# Autodesk Inventor assembly: Layout Test Assembly
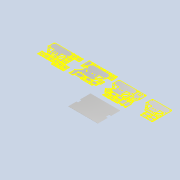
[picture p0: Inventor's stored thumbnail of the model, 180x180]
Saved by Autodesk Inventor 2022 (Build 260153000, 153)
## iProperties
Created: 2021-10-30
Part Number: Layout Test Assembly
Document SubType Name: Assembly
Designer: Coy
Author: Coy
## Documents named in this file (12)
- H:\3D Files\Project 3D Models\Breakfast Maker 2000\Machined Parts\Layout Test Assembly.iam
- H:\3D Files\Project 3D Models\Breakfast Maker 2000\Machined Parts\Stock Aluminum Sheet.ipt
- H:\3D Files\Project 3D Models\Breakfast Maker 2000\Machined Parts\X Axis Belt Motor Inside Frame Machined.ipt
- H:\3D Files\Project 3D Models\Breakfast Maker 2000\Machined Parts\X Axis Belt V Wheel and Motor Frame Machined.ipt
- H:\3D Files\Project 3D Models\Breakfast Maker 2000\Machined Parts\X Axis Belt V Wheel Frame Machined.ipt
- H:\3D Files\Project 3D Models\Breakfast Maker 2000\Machined Parts\X Axis Belt V Wheel LEFT Outside Frame Machined.ipt
- H:\3D Files\Project 3D Models\Breakfast Maker 2000\Machined Parts\X Axis Belt V Wheel RIGHT Outside Frame Machined.ipt
- H:\3D Files\Project 3D Models\Breakfast Maker 2000\Machined Parts\2x4 2020 Extrusion Gusset Connector.ipt
- H:\3D Files\Project 3D Models\Breakfast Maker 2000\Machined Parts\X Axis Statonary Composite Belt Holder.ipt
- H:\3D Files\Project 3D Models\Breakfast Maker 2000\Machined Parts\X Axis Statonary NON ADJUSTABLE Composite Belt Holder.ipt
- H:\3D Files\Project 3D Models\Breakfast Maker 2000\Machined Parts\X Axis Drag Chain 2020 Connecting Bracket.ipt
- H:\3D Files\Project 3D Models\Breakfast Maker 2000\Machined Parts\Generic 3x3 Corner Connecting Gusset.ipt
## Components (34 placed, 11 different names)
1. Stock Aluminum Sheet:1 — Mate:1, Mate:2, Mate:3, Mate:4, Mate:5, Mate:6, Mate:7, Mate:8, Mate:9, Mate:10, Mate:11, Mate:12, Mate:13, Mate:14, Mate:15, Mate:16, Mate:17, Mate:18, Mate:19, Mate:20, Mate:22, Mate:23, Mate:24, Mate:26, Mate:28, Mate:29, Mate:30, Mate:31, Mate:42, Mate:54, Mate:55, Mate:84, Mate:85
2. X Axis Belt Motor Inside Frame Machined:1 — Mate:54, Mate:56, Flush:4, Mate:67
3. X Axis Belt V Wheel and Motor Frame Machined:1 — Mate:4, Mate:68, Flush:10, Flush:15, Mate:78, Mate:83
4. X Axis Belt V Wheel Frame Machined:1 — Mate:3, Mate:80, Mate:86, Flush:20
5. X Axis Belt V Wheel LEFT Outside Frame Machined:1 — Mate:2, Mate:56, Flush:4, Mate:57, Mate:58, Mate:64, Mate:81
6. X Axis Belt V Wheel RIGHT Outside Frame Machined:1 — Mate:1, Mate:43, Mate:44, Mate:45, Mate:46, Mate:48, Mate:51, Flush:2, Mate:52, Flush:3, Tangent:1, Mate:82
7. 2x4 2020 Extrusion Gusset Connector:1 — Mate:22, Mate:58, Mate:59, Mate:60, Mate:61, Mate:64, Tangent:3, Mate:65
8. 2x4 2020 Extrusion Gusset Connector:2 — Mate:23, Mate:47, Mate:48, Mate:49, Mate:50
9. X Axis Statonary Composite Belt Holder:1 — Mate:55, Mate:66, Flush:5
10. X Axis Statonary Composite Belt Holder:2 — Mate:24, Mate:65, Mate:66, Flush:5, Mate:67
11. X Axis Statonary NON ADJUSTABLE Composite Belt Holder:1 — Mate:26, Mate:43, Flush:1
12. X Axis Statonary NON ADJUSTABLE Composite Belt Holder:2 — Mate:42, Mate:45, Mate:46, Mate:47, Tangent:2
13. X Axis Drag Chain 2020 Connecting Bracket:1 — Mate:28, Mate:44, Flush:1, Flush:3, Mate:53
14. X Axis Drag Chain 2020 Connecting Bracket:2 — Mate:30, Mate:52, Mate:53
15. X Axis Drag Chain 2020 Connecting Bracket:3 — Mate:29, Mate:79, Flush:18
16. X Axis Drag Chain 2020 Connecting Bracket:4 — Mate:31, Mate:49, Tangent:2
17. Generic 3x3 Corner Connecting Gusset:1 — Mate:17, Mate:57, Tangent:3, Tangent:4
18. Generic 3x3 Corner Connecting Gusset:2 — Mate:18, Flush:12, Mate:75, Flush:17, Mate:77
19. Generic 3x3 Corner Connecting Gusset:3 — Mate:19, Flush:7, Flush:8, Mate:68, Mate:71, Mate:72
20. Generic 3x3 Corner Connecting Gusset:4 — Mate:20, Flush:6, Mate:70
21. Generic 3x3 Corner Connecting Gusset:5 — Mate:13, Flush:17, Mate:77, Mate:79, Flush:18
22. Generic 3x3 Corner Connecting Gusset:6 — Mate:14, Flush:16, Mate:76
23. Generic 3x3 Corner Connecting Gusset:7 — Mate:15, Mate:61, Mate:63
24. Generic 3x3 Corner Connecting Gusset:8 — Mate:16, Mate:51, Flush:2
25. Generic 3x3 Corner Connecting Gusset:9 — Mate:9, Flush:8, Mate:72, Flush:10
26. Generic 3x3 Corner Connecting Gusset:10 — Mate:10, Flush:13, Flush:14, Mate:73, Mate:74, Mate:78
27. Generic 3x3 Corner Connecting Gusset:11 — Mate:11, Flush:6, Flush:7, Mate:70, Mate:71
28. Generic 3x3 Corner Connecting Gusset:12 — Mate:12, Mate:50, Tangent:1
29. Generic 3x3 Corner Connecting Gusset:13 — Mate:5, Mate:60, Mate:62, Mate:63
30. Generic 3x3 Corner Connecting Gusset:14 — Mate:6, Mate:59, Mate:62, Tangent:4
31. Generic 3x3 Corner Connecting Gusset:15 — Mate:7, Flush:14, Mate:73, Flush:15, Flush:16, Mate:76
32. Generic 3x3 Corner Connecting Gusset:16 — Mate:8, Flush:12, Flush:13, Mate:74, Mate:75
33. 2x4 2020 Extrusion Gusset Connector:3 — Mate:85, Mate:87, Flush:19
34. 2x4 2020 Extrusion Gusset Connector:4 — Mate:84, Mate:86, Mate:87, Flush:19, Flush:20
## Relationships (95: Mate 73, Flush 18, Tangent 4)
- Mate:1: Stock Aluminum Sheet:1 ↔ X Axis Belt V Wheel RIGHT Outside Frame Machined:1
- Mate:2: Stock Aluminum Sheet:1 ↔ X Axis Belt V Wheel LEFT Outside Frame Machined:1
- Mate:3: Stock Aluminum Sheet:1 ↔ X Axis Belt V Wheel Frame Machined:1
- Mate:4: Stock Aluminum Sheet:1 ↔ X Axis Belt V Wheel and Motor Frame Machined:1
- Mate:5: Stock Aluminum Sheet:1 ↔ Generic 3x3 Corner Connecting Gusset:13
- Mate:6: Stock Aluminum Sheet:1 ↔ Generic 3x3 Corner Connecting Gusset:14
- Mate:7: Stock Aluminum Sheet:1 ↔ Generic 3x3 Corner Connecting Gusset:15
- Mate:8: Stock Aluminum Sheet:1 ↔ Generic 3x3 Corner Connecting Gusset:16
- Mate:9: Stock Aluminum Sheet:1 ↔ Generic 3x3 Corner Connecting Gusset:9
- Mate:10: Stock Aluminum Sheet:1 ↔ Generic 3x3 Corner Connecting Gusset:10
- Mate:11: Stock Aluminum Sheet:1 ↔ Generic 3x3 Corner Connecting Gusset:11
- Mate:12: Stock Aluminum Sheet:1 ↔ Generic 3x3 Corner Connecting Gusset:12
- Mate:13: Stock Aluminum Sheet:1 ↔ Generic 3x3 Corner Connecting Gusset:5
- Mate:14: Stock Aluminum Sheet:1 ↔ Generic 3x3 Corner Connecting Gusset:6
- Mate:15: Stock Aluminum Sheet:1 ↔ Generic 3x3 Corner Connecting Gusset:7
- Mate:16: Stock Aluminum Sheet:1 ↔ Generic 3x3 Corner Connecting Gusset:8
- Mate:17: Stock Aluminum Sheet:1 ↔ Generic 3x3 Corner Connecting Gusset:1
- Mate:18: Stock Aluminum Sheet:1 ↔ Generic 3x3 Corner Connecting Gusset:2
- Mate:19: Stock Aluminum Sheet:1 ↔ Generic 3x3 Corner Connecting Gusset:3
- Mate:20: Stock Aluminum Sheet:1 ↔ Generic 3x3 Corner Connecting Gusset:4
- Mate:22: Stock Aluminum Sheet:1 ↔ 2x4 2020 Extrusion Gusset Connector:1
- Mate:23: Stock Aluminum Sheet:1 ↔ 2x4 2020 Extrusion Gusset Connector:2
- Mate:24: Stock Aluminum Sheet:1 ↔ X Axis Statonary Composite Belt Holder:2
- Mate:26: Stock Aluminum Sheet:1 ↔ X Axis Statonary NON ADJUSTABLE Composite Belt Holder:1
- Mate:28: Stock Aluminum Sheet:1 ↔ X Axis Drag Chain 2020 Connecting Bracket:1
- Mate:29: Stock Aluminum Sheet:1 ↔ X Axis Drag Chain 2020 Connecting Bracket:3
- Mate:30: Stock Aluminum Sheet:1 ↔ X Axis Drag Chain 2020 Connecting Bracket:2
- Mate:31: Stock Aluminum Sheet:1 ↔ X Axis Drag Chain 2020 Connecting Bracket:4
- Mate:42: Stock Aluminum Sheet:1 ↔ X Axis Statonary NON ADJUSTABLE Composite Belt Holder:2
- Mate:43 (3.175 mm): X Axis Belt V Wheel RIGHT Outside Frame Machined:1 ↔ X Axis Statonary NON ADJUSTABLE Composite Belt Holder:1
- Mate:44 (3.175 mm): X Axis Belt V Wheel RIGHT Outside Frame Machined:1 ↔ X Axis Drag Chain 2020 Connecting Bracket:1
- Flush:1: X Axis Statonary NON ADJUSTABLE Composite Belt Holder:1 ↔ X Axis Drag Chain 2020 Connecting Bracket:1
- Mate:45 (3.175 mm): X Axis Belt V Wheel RIGHT Outside Frame Machined:1 ↔ X Axis Statonary NON ADJUSTABLE Composite Belt Holder:2
- Mate:46 (3.175 mm): X Axis Belt V Wheel RIGHT Outside Frame Machined:1 ↔ X Axis Statonary NON ADJUSTABLE Composite Belt Holder:2
- Mate:47 (3.175 mm): 2x4 2020 Extrusion Gusset Connector:2 ↔ X Axis Statonary NON ADJUSTABLE Composite Belt Holder:2
- Mate:48 (3.175 mm): X Axis Belt V Wheel RIGHT Outside Frame Machined:1 ↔ 2x4 2020 Extrusion Gusset Connector:2
- Mate:49 (3.175 mm): 2x4 2020 Extrusion Gusset Connector:2 ↔ X Axis Drag Chain 2020 Connecting Bracket:4
- Mate:50 (3.175 mm): 2x4 2020 Extrusion Gusset Connector:2 ↔ Generic 3x3 Corner Connecting Gusset:12
- Mate:51 (3.175 mm): X Axis Belt V Wheel RIGHT Outside Frame Machined:1 ↔ Generic 3x3 Corner Connecting Gusset:8
- Flush:2: X Axis Belt V Wheel RIGHT Outside Frame Machined:1 ↔ Generic 3x3 Corner Connecting Gusset:8
- Mate:52 (3.175 mm): X Axis Belt V Wheel RIGHT Outside Frame Machined:1 ↔ X Axis Drag Chain 2020 Connecting Bracket:2
- Flush:3: X Axis Belt V Wheel RIGHT Outside Frame Machined:1 ↔ X Axis Drag Chain 2020 Connecting Bracket:1
- Mate:53 (3.175 mm): X Axis Drag Chain 2020 Connecting Bracket:1 ↔ X Axis Drag Chain 2020 Connecting Bracket:2
- Tangent:1 (3.175 mm): X Axis Belt V Wheel RIGHT Outside Frame Machined:1 ↔ Generic 3x3 Corner Connecting Gusset:12
- Tangent:2 (3.175 mm): X Axis Statonary NON ADJUSTABLE Composite Belt Holder:2 ↔ X Axis Drag Chain 2020 Connecting Bracket:4
- Mate:54: Stock Aluminum Sheet:1 ↔ X Axis Belt Motor Inside Frame Machined:1
- Mate:55: Stock Aluminum Sheet:1 ↔ X Axis Statonary Composite Belt Holder:1
- Mate:56 (3.175 mm): X Axis Belt Motor Inside Frame Machined:1 ↔ X Axis Belt V Wheel LEFT Outside Frame Machined:1
- Flush:4: X Axis Belt Motor Inside Frame Machined:1 ↔ X Axis Belt V Wheel LEFT Outside Frame Machined:1
- Mate:57 (3.175 mm): X Axis Belt V Wheel LEFT Outside Frame Machined:1 ↔ Generic 3x3 Corner Connecting Gusset:1
- Mate:58 (3.175 mm): X Axis Belt V Wheel LEFT Outside Frame Machined:1 ↔ 2x4 2020 Extrusion Gusset Connector:1
- Mate:59 (3.175 mm): 2x4 2020 Extrusion Gusset Connector:1 ↔ Generic 3x3 Corner Connecting Gusset:14
- Mate:60 (3.175 mm): 2x4 2020 Extrusion Gusset Connector:1 ↔ Generic 3x3 Corner Connecting Gusset:13
- Mate:61 (3.175 mm): 2x4 2020 Extrusion Gusset Connector:1 ↔ Generic 3x3 Corner Connecting Gusset:7
- Mate:62 (3.175 mm): Generic 3x3 Corner Connecting Gusset:13 ↔ Generic 3x3 Corner Connecting Gusset:14
- Mate:63 (3.175 mm): Generic 3x3 Corner Connecting Gusset:7 ↔ Generic 3x3 Corner Connecting Gusset:13
- Mate:64: X Axis Belt V Wheel LEFT Outside Frame Machined:1 ↔ 2x4 2020 Extrusion Gusset Connector:1
- Tangent:3 (3.175 mm): 2x4 2020 Extrusion Gusset Connector:1 ↔ Generic 3x3 Corner Connecting Gusset:1
- Tangent:4 (3.175 mm): Generic 3x3 Corner Connecting Gusset:1 ↔ Generic 3x3 Corner Connecting Gusset:14
- Mate:65 (3.175 mm): 2x4 2020 Extrusion Gusset Connector:1 ↔ X Axis Statonary Composite Belt Holder:2
- Mate:66 (3.175 mm): X Axis Statonary Composite Belt Holder:1 ↔ X Axis Statonary Composite Belt Holder:2
- Flush:5: X Axis Statonary Composite Belt Holder:1 ↔ X Axis Statonary Composite Belt Holder:2
- Mate:67 (3.175 mm): X Axis Belt Motor Inside Frame Machined:1 ↔ X Axis Statonary Composite Belt Holder:2
- Flush:6: Generic 3x3 Corner Connecting Gusset:4 ↔ Generic 3x3 Corner Connecting Gusset:11
- Flush:7: Generic 3x3 Corner Connecting Gusset:3 ↔ Generic 3x3 Corner Connecting Gusset:11
- Flush:8: Generic 3x3 Corner Connecting Gusset:3 ↔ Generic 3x3 Corner Connecting Gusset:9
- Mate:68 (3.175 mm): X Axis Belt V Wheel and Motor Frame Machined:1 ↔ Generic 3x3 Corner Connecting Gusset:3
- Mate:70 (3.175 mm): Generic 3x3 Corner Connecting Gusset:4 ↔ Generic 3x3 Corner Connecting Gusset:11
- Mate:71 (3.175 mm): Generic 3x3 Corner Connecting Gusset:3 ↔ Generic 3x3 Corner Connecting Gusset:11
- Mate:72 (3.175 mm): Generic 3x3 Corner Connecting Gusset:3 ↔ Generic 3x3 Corner Connecting Gusset:9
- Flush:10: X Axis Belt V Wheel and Motor Frame Machined:1 ↔ Generic 3x3 Corner Connecting Gusset:9
- Flush:12: Generic 3x3 Corner Connecting Gusset:2 ↔ Generic 3x3 Corner Connecting Gusset:16
- Flush:13: Generic 3x3 Corner Connecting Gusset:10 ↔ Generic 3x3 Corner Connecting Gusset:16
- Flush:14: Generic 3x3 Corner Connecting Gusset:10 ↔ Generic 3x3 Corner Connecting Gusset:15
- Mate:73 (3.175 mm): Generic 3x3 Corner Connecting Gusset:10 ↔ Generic 3x3 Corner Connecting Gusset:15
- Mate:74 (3.175 mm): Generic 3x3 Corner Connecting Gusset:10 ↔ Generic 3x3 Corner Connecting Gusset:16
- Mate:75 (3.175 mm): Generic 3x3 Corner Connecting Gusset:2 ↔ Generic 3x3 Corner Connecting Gusset:16
- Flush:15: X Axis Belt V Wheel and Motor Frame Machined:1 ↔ Generic 3x3 Corner Connecting Gusset:15
- Flush:16: Generic 3x3 Corner Connecting Gusset:6 ↔ Generic 3x3 Corner Connecting Gusset:15
- Mate:76 (3.175 mm): Generic 3x3 Corner Connecting Gusset:6 ↔ Generic 3x3 Corner Connecting Gusset:15
- Flush:17: Generic 3x3 Corner Connecting Gusset:2 ↔ Generic 3x3 Corner Connecting Gusset:5
- Mate:77 (3.175 mm): Generic 3x3 Corner Connecting Gusset:2 ↔ Generic 3x3 Corner Connecting Gusset:5
- Mate:78 (3.175 mm): X Axis Belt V Wheel and Motor Frame Machined:1 ↔ Generic 3x3 Corner Connecting Gusset:10
- Mate:79 (3.175 mm): X Axis Drag Chain 2020 Connecting Bracket:3 ↔ Generic 3x3 Corner Connecting Gusset:5
- Flush:18: X Axis Drag Chain 2020 Connecting Bracket:3 ↔ Generic 3x3 Corner Connecting Gusset:5
- Mate:80 (-500 mm): X Axis Belt V Wheel Frame Machined:1
- Mate:81 (-500 mm): X Axis Belt V Wheel LEFT Outside Frame Machined:1
- Mate:82 (-500 mm): X Axis Belt V Wheel RIGHT Outside Frame Machined:1
- Mate:83 (-500 mm): X Axis Belt V Wheel and Motor Frame Machined:1
- Mate:84: Stock Aluminum Sheet:1 ↔ 2x4 2020 Extrusion Gusset Connector:4
- Mate:85: Stock Aluminum Sheet:1 ↔ 2x4 2020 Extrusion Gusset Connector:3
- Mate:86 (3.175 mm): X Axis Belt V Wheel Frame Machined:1 ↔ 2x4 2020 Extrusion Gusset Connector:4
- Mate:87 (3.175 mm): 2x4 2020 Extrusion Gusset Connector:3 ↔ 2x4 2020 Extrusion Gusset Connector:4
- Flush:19: 2x4 2020 Extrusion Gusset Connector:3 ↔ 2x4 2020 Extrusion Gusset Connector:4
- Flush:20: X Axis Belt V Wheel Frame Machined:1 ↔ 2x4 2020 Extrusion Gusset Connector:4
